# Autodesk Inventor assembly: MotorModule
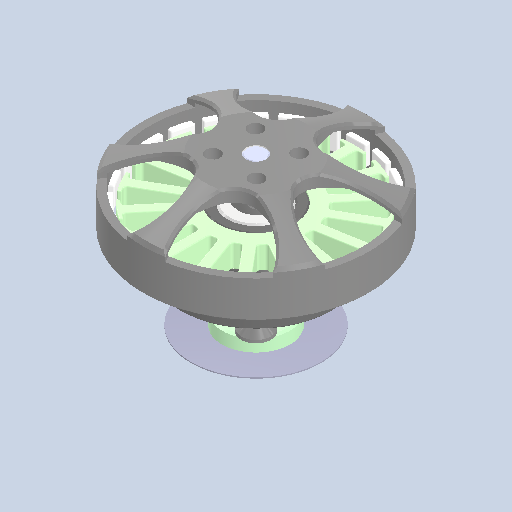
[picture p0: Inventor's stored thumbnail of the model, 512x512]
Saved by Autodesk Inventor 2023 (Build 270158000, 158)
## iProperties
Created: 2016-08-15
Part Number: MotorModule
Document SubType Name: Assembly
Designer: Jochen
Sending System: SolidWorks 2017
Last Author: Felix
Last Saved: 2021-02-23
Author: Jochen
## Documents named in this file (7)
- D:\Projects\Lisbeth\CAD\Common\Motor\MotorModule.iam
- D:\Projects\Lisbeth\CAD\Tools\Motor Testbed\motor_antigravity_4004_custom_shaft.iam
- D:\Projects\Lisbeth\CAD\Common\Encoder\encoder_codewheel_5000cpr_pwb_7mm.ipt
- D:\Projects\Lisbeth\CAD\Common\Bearing\bearing_8_4_2_sbn_MR84VA.ipt
- D:\Projects\Lisbeth\CAD\Common\Fastener\fastener_fhs_m3_5.ipt
- D:\Projects\Lisbeth\CAD\Common\Pulley\MotorPulley.ipt
- D:\Projects\Lisbeth\CAD\Common\Encoder\EncoderCodeWheelMount T2.5.ipt
## Components (9 placed, 6 different names)
1. motor_antigravity_4004_custom_shaft:2 [sub-assembly] — Mate:32, Mate:33, Mate:34, Mate:35
2. encoder_codewheel_5000cpr_pwb_7mm:1 — Mate:20, Mate:26
3. bearing_8_4_2_sbn_MR84VA:1 — Mate:29, Mate:35
4. fastener_fhs_m3_5:3
5. fastener_fhs_m3_5:1
6. fastener_fhs_m3_5:4
7. fastener_fhs_m3_5:2
8. TransmissionPulleyMotor:1 — Mate:22, Mate:32, Mate:33
9. EncoderWheelMount T2.5:1 — Mate:20, Mate:22, Mate:26, Mate:29, Mate:34
## Relationships (8: Mate 8)
- Mate:20: encoder_codewheel_5000cpr_pwb_7mm:1 ↔ EncoderWheelMount T2.5:1
- Mate:22 (0.3 mm): TransmissionPulleyMotor:1 ↔ EncoderWheelMount T2.5:1
- Mate:26: encoder_codewheel_5000cpr_pwb_7mm:1 ↔ EncoderWheelMount T2.5:1
- Mate:29: bearing_8_4_2_sbn_MR84VA:1 ↔ EncoderWheelMount T2.5:1
- Mate:32 (0.6 mm): motor_antigravity_4004_custom_shaft:2 ↔ TransmissionPulleyMotor:1
- Mate:33: motor_antigravity_4004_custom_shaft:2 ↔ TransmissionPulleyMotor:1
- Mate:34: motor_antigravity_4004_custom_shaft:2 ↔ EncoderWheelMount T2.5:1
- Mate:35: motor_antigravity_4004_custom_shaft:2 ↔ bearing_8_4_2_sbn_MR84VA:1
